# Autodesk Inventor assembly: Assembly1
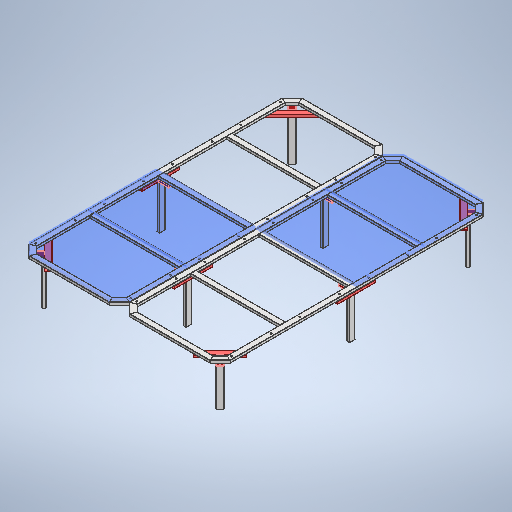
[picture p0: Inventor's stored thumbnail of the model, 512x512]
Saved by Autodesk Inventor 2026.2 (Build 302298000, 298)
## iProperties
Created: 2026-05-20
Part Number: Assembly1
Document SubType Name: Assembly
Designer: admin
Author: admin
## Documents named in this file (2)
- C:\Users\admin\Documents\Inventor\Debbed\Assembly1.iam
- C:\Users\admin\Documents\Inventor\Debbed\Assembly2.iam
## Components (2 placed, 1 different names)
1. Assembly2:1 [sub-assembly] — Rigid:1
2. Assembly2:2 [sub-assembly] — Rigid:1
## Relationships (1: WeldJoint 1)
- Rigid:1 [WeldJoint]: Assembly2:1 ↔ Assembly2:2
